# Autodesk Inventor assembly: The Final Assembly
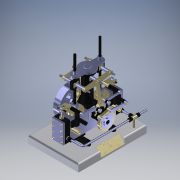
[picture p0: Inventor's stored thumbnail of the model, 180x180]
Saved by Autodesk Inventor 2016 SP1 (Build 200210100, 210)
## iProperties
Created: 2016-12-03
Part Number: The Final Assembly
Document SubType Name: Assembly
Designer: Muhammad
Author: Muhammad
## Documents named in this file (45)
- E:\Brenays Steam Engine, USB\The Final Assembly.iam
- E:\Brenays Steam Engine, USB\Base.ipt
- E:\Brenays Steam Engine, USB\Etichetta.ipt
- E:\Brenays Steam Engine, USB\Coperchio inferiore.ipt
- E:\Brenays Steam Engine, USB\Carcassa.ipt
- E:\Brenays Steam Engine, USB\Distributore.ipt
- E:\Brenays Steam Engine, USB\Coperchio.ipt
- E:\Brenays Steam Engine, USB\Premistoppa M10x1.ipt
- E:\Brenays Steam Engine, USB\Albero a gomito.ipt
- E:\Brenays Steam Engine, USB\Guida testa a croce.ipt
- E:\Brenays Steam Engine, USB\Coperchio Superiore.ipt
- E:\Brenays Steam Engine, USB\Supporto SX.ipt
- E:\Brenays Steam Engine, USB\Supporto DX.ipt
- E:\Brenays Steam Engine, USB\Asta cassetto.ipt
- E:\Brenays Steam Engine, USB\Cassetto.ipt
- E:\Brenays Steam Engine, USB\Fermo 5 mm.ipt
- E:\Brenays Steam Engine, USB\Asta cassetto_MIR.ipt
- E:\Brenays Steam Engine, USB\Cassetto_MIR.ipt
- E:\Brenays Steam Engine, USB\Fermo 5 mm_MIR.ipt
- E:\Brenays Steam Engine, USB\Biella.ipt
- E:\Brenays Steam Engine, USB\Bielletta.ipt
- E:\Brenays Steam Engine, USB\Spina cilindrica.ipt
- E:\Brenays Steam Engine, USB\Manovella.ipt
- E:\Brenays Steam Engine, USB\Assieme eccentrico.ipt
- E:\Brenays Steam Engine, USB\Testata Superiore.ipt
- E:\Brenays Steam Engine, USB\Premistoppa.ipt
- E:\Brenays Steam Engine, USB\Asta pistone.ipt
- E:\Brenays Steam Engine, USB\T di connessione1.ipt
- E:\Brenays Steam Engine, USB\Semi albero F.ipt
- E:\Brenays Steam Engine, USB\Semi alberto M.ipt
- E:\Brenays Steam Engine, USB\Traversa.ipt
- E:\Brenays Steam Engine, USB\Cursore.ipt
- E:\Brenays Steam Engine, USB\Spina cilindrica4.ipt
- E:\Brenays Steam Engine, USB\Forcella.ipt
- E:\Brenays Steam Engine, USB\Volano.ipt
- E:\Brenays Steam Engine, USB\Semi Cuscinetto.ipt
- E:\Brenays Steam Engine, USB\Varia.ipt
- E:\Brenays Steam Engine, USB\Inlet Pipe Nipple.ipt
- E:\Brenays Steam Engine, USB\Tube.ipt
- E:\Brenays Steam Engine, USB\Steam Inlet Pipe 1.ipt
- E:\Brenays Steam Engine, USB\Steam Inlet T Connector.ipt
- E:\Brenays Steam Engine, USB\M8x6 Pipe Nut.ipt
- E:\Brenays Steam Engine, USB\Exhaust Pipe Connector.ipt
- E:\Brenays Steam Engine, USB\Nut.ipt
- E:\Brenays Steam Engine, USB\Nut_MIR.ipt
## Components (93 placed, 44 different names)
1. Base:1 — Rigid:1, Rigid:2, Rigid:3, Flush:7
2. Etichetta:1 — Rigid:1
3. Coperchio inferiore:1 — Rigid:2
4. Coperchio inferiore:2 — Rigid:3, Rigid:4
5. Carcassa:1 — Rigid:4, Rigid:5, Rigid:6, Rotational:1, Rigid:11, Rigid:13, Rigid:14, Rigid:20, Rigid:21, Rigid:37, Rigid:38
6. Distributore:1 — Rigid:5, Rigid:8, Rigid:9, Rigid:26
7. Distributore:2 — Rigid:6, Rigid:7, Rigid:10, Angle:1, Mate:5, Rigid:27
8. Coperchio:1 — Rigid:7, Rigid:45, Rigid:46, Rigid:47, Rigid:48, Rigid:49, Rigid:50, Rigid:51, Rigid:52
9. Coperchio:2 — Rigid:8
10. Premistoppa M10x1:1 — Rigid:9, Mate:9
11. Premistoppa M10x1:2 — Rigid:10, Mate:1
12. Albero a gomito:1 — Rotational:1, Mate:18, Flush:4, Angle:2, Mate:28, Mate:29, Mate:30, Mate:31, Rigid:24, Mate:45, Mate:46, Mate:48, Mate:49
13. Guida testa a croce:1 — Rigid:11, Rigid:12, Mate:40
14. Coperchio Superiore:1 — Rigid:12, Mate:26, Mate:27
15. Supporto SX:1 — Rigid:14, Mate:23, Mate:55, Mate:56
16. Supporto DX:1 — Rigid:13, Rigid:19, Mate:17, Mate:24, Rotational:2
17. Asta cassetto:1 — Mate:1, Mate:4, Flush:1, Mate:44
18. Cassetto:1 — Mate:2, Rigid:15, Mate:3, Rigid:16, Angle:1, Mate:5
19. Fermo 5 mm:1 — Mate:2, Rigid:15, Mate:4
20. Fermo 5 mm:2 — Mate:3, Rigid:16, Flush:1
21. Asta cassetto_MIR:1 — Mate:6, Flush:3, Mate:9, Rigid:25
22. Cassetto_MIR:1 — Mate:7, Mate:8, Rigid:17, Rigid:18
23. Fermo 5 mm_MIR:1 — Mate:6, Mate:7, Rigid:17
24. Fermo 5 mm_MIR:2 — Flush:3, Mate:8, Rigid:18
25. Biella:1 — Mate:10, Mate:11, Mate:12, Rigid:43
26. Biella:2 — Mate:15, Mate:16, Mate:17, Mate:24, Angle:7, Rigid:44
27. Bielletta:1 — Mate:13, Mate:14, Mate:15, Mate:16, Rigid:36
28. Bielletta:2 — Mate:19, Mate:20, Mate:21, Mate:22, Rotational:4
29. Spina cilindrica:1 — Rigid:19, Mate:12
30. Assieme eccentrico:1 — Mate:18, Flush:4, Mate:25, Angle:2
31. Manovella:1 — Mate:10, Mate:11, Mate:13, Mate:14, Mate:19, Mate:20, Mate:25, Rigid:35
32. Biella:3 — Mate:21, Mate:22, Mate:23, Angle:8, Rigid:41
33. Testata Superiore:1 — Rigid:21, Rigid:23
34. Testata Superiore:2 — Rigid:20, Rigid:22
35. Premistoppa:1 — Rigid:23
36. Premistoppa:2 — Rigid:22
37. Asta pistone:1 — Mate:26, Angle:4, Angle:5, Mate:52, Flush:5
38. Asta pistone:2 — Mate:27, Angle:4, Mate:54, Flush:6
39. T di connessione1:1 — Mate:28, Mate:29, Mate:32, Angle:3, Mate:35, Mate:36, Mate:37, Angle:5, Mate:41, Mate:42, Mate:47
40. T di connessione1:2 — Mate:30, Mate:31, Mate:33, Angle:3, Mate:34, Mate:38, Mate:39, Mate:50
41. Semi albero F:1 — Mate:33, Mate:34
42. Semi alberto M:1 — Mate:32, Mate:35, Mate:51
43. Semi alberto M:2 — Mate:36, Mate:37, Mate:53
44. Semi albero F:2 — Mate:38, Mate:39
45. Traversa:1 — Mate:41, Mate:42, Mate:43
46. Cursore:1 — Mate:40, Mate:43
47. Spina cilindrica4:1 — Mate:44, Angle:6
48. Forcella:1 — Rotational:2, Angle:6, Angle:7
49. Volano:1 — Rigid:24
50. Semi Cuscinetto:1 — Mate:45, Mate:46, Mate:47
51. Semi Cuscinetto:2 — Mate:48, Mate:49, Mate:50
52. Varia:1 — Mate:51, Mate:52, Flush:5
53. Varia:2 — Mate:53, Mate:54, Flush:6
54. Forcella:2 — Mate:55, Mate:56, Angle:8
55. Spina cilindrica4:2 — Rigid:25
56. Inlet Pipe Nipple:1 — Rigid:26, Rotational:3, Rigid:30
57. Inlet Pipe Nipple:2 — Rigid:27, Rigid:28, Rigid:33
58. Tube:1 — Rotational:3, Mate:57
59. Steam Inlet Pipe 1:1 — Rigid:28, Mate:58
60. Steam Inlet T Connector:1 — Mate:57, Mate:58, Rigid:29, Rigid:31, Rigid:32, Rigid:34
61. Steam Inlet Pipe 1:2 — Rigid:29
62. M8x6 Pipe Nut:1 — Rigid:34
63. M8x6 Pipe Nut:2 — Rigid:32
64. M8x6 Pipe Nut:3 — Rigid:31
65. M8x6 Pipe Nut:4 — Rigid:30
66. M8x6 Pipe Nut:5 — Rigid:33
67. Fermo 5 mm:3 — Rigid:35, Rigid:42
68. Fermo 5 mm:4 — Rotational:4, Rigid:40
69. Fermo 5 mm:5 — Rigid:36, Rigid:39
70. Exhaust Pipe Connector:1 — Rigid:37
71. Exhaust Pipe Connector:2 — Rigid:38
72. Spina cilindrica:2 — Rigid:39
73. Spina cilindrica:3 — Rigid:41
74. Spina cilindrica:4 — Rigid:40
75. Spina cilindrica:5 — Rigid:43
76. Spina cilindrica:6 — Rigid:42
77. Spina cilindrica:7 — Rigid:44
78. Nut:6 — Rigid:45
79. Nut:7 — Rigid:46
80. Nut:8 — Rigid:47
81. Nut:9 — Rigid:48
82. Nut:10 — Rigid:49
83. Nut:11 — Rigid:50
84. Nut:12 — Rigid:51
85. Nut:13 — Rigid:52
86. Nut_MIR:1
87. Nut_MIR:2
88. Nut_MIR:3
89. Nut_MIR:4
90. Nut_MIR:5
91. Nut_MIR:6
92. Nut_MIR:7
93. Nut_MIR:8
## Relationships (129: Mate 58, WeldJoint 52, Angle 8, Flush 7, RevoluteJoint 4)
- Rigid:1 [WeldJoint]: Base:1 ↔ Etichetta:1
- Rigid:2 [WeldJoint]: Base:1 ↔ Coperchio inferiore:1
- Rigid:3 [WeldJoint]: Base:1 ↔ Coperchio inferiore:2
- Rigid:4 [WeldJoint]: Coperchio inferiore:2 ↔ Carcassa:1
- Rigid:5 [WeldJoint]: Carcassa:1 ↔ Distributore:1
- Rigid:6 [WeldJoint]: Carcassa:1 ↔ Distributore:2
- Rigid:7 [WeldJoint]: Distributore:2 ↔ Coperchio:1
- Rigid:8 [WeldJoint]: Distributore:1 ↔ Coperchio:2
- Rigid:9 [WeldJoint]: Distributore:1 ↔ Premistoppa M10x1:1
- Rigid:10 [WeldJoint]: Distributore:2 ↔ Premistoppa M10x1:2
- Rotational:1 [RevoluteJoint]: Carcassa:1 ↔ Albero a gomito:1
- Rigid:11 [WeldJoint]: Carcassa:1 ↔ Guida testa a croce:1
- Rigid:12 [WeldJoint]: Guida testa a croce:1 ↔ Coperchio Superiore:1
- Rigid:13 [WeldJoint]: Carcassa:1 ↔ Supporto DX:1
- Rigid:14 [WeldJoint]: Carcassa:1 ↔ Supporto SX:1
- Mate:1: Premistoppa M10x1:2 ↔ Asta cassetto:1
- Mate:2: Cassetto:1 ↔ Fermo 5 mm:1
- Rigid:15 [WeldJoint]: Cassetto:1 ↔ Fermo 5 mm:1
- Mate:3: Cassetto:1 ↔ Fermo 5 mm:2
- Rigid:16 [WeldJoint]: Cassetto:1 ↔ Fermo 5 mm:2
- Mate:4: Asta cassetto:1 ↔ Fermo 5 mm:1
- Angle:1 (0 deg): Distributore:2 ↔ Cassetto:1
- Mate:5: Distributore:2 ↔ Cassetto:1
- Flush:1 (1.7 mm): Asta cassetto:1 ↔ Fermo 5 mm:2
- Flush:2
- Mate:6: Asta cassetto_MIR:1 ↔ Fermo 5 mm_MIR:1
- Mate:7: Cassetto_MIR:1 ↔ Fermo 5 mm_MIR:1
- Flush:3 (1.7 mm): Asta cassetto_MIR:1 ↔ Fermo 5 mm_MIR:2
- Mate:8: Cassetto_MIR:1 ↔ Fermo 5 mm_MIR:2
- Rigid:17 [WeldJoint]: Cassetto_MIR:1 ↔ Fermo 5 mm_MIR:1
- Rigid:18 [WeldJoint]: Cassetto_MIR:1 ↔ Fermo 5 mm_MIR:2
- Mate:9: Premistoppa M10x1:1 ↔ Asta cassetto_MIR:1
- Rigid:19 [WeldJoint]: Supporto DX:1 ↔ Spina cilindrica:1
- Mate:10: Biella:1 ↔ Manovella:1
- Mate:11: Biella:1 ↔ Manovella:1
- Mate:12: Biella:1 ↔ Spina cilindrica:1
- Mate:13: Bielletta:1 ↔ Manovella:1
- Mate:14: Bielletta:1 ↔ Manovella:1
- Mate:15: Biella:2 ↔ Bielletta:1
- Mate:16: Biella:2 ↔ Bielletta:1
- Mate:17: Supporto DX:1 ↔ Biella:2
- Mate:18: Albero a gomito:1 ↔ Assieme eccentrico:1
- Mate:19: Bielletta:2 ↔ Manovella:1
- Mate:20: Bielletta:2 ↔ Manovella:1
- Mate:21: Bielletta:2 ↔ Biella:3
- Mate:22: Bielletta:2 ↔ Biella:3
- Mate:23: Supporto SX:1 ↔ Biella:3
- Mate:24: Supporto DX:1 ↔ Biella:2
- Flush:4: Albero a gomito:1 ↔ Assieme eccentrico:1
- Mate:25: Assieme eccentrico:1 ↔ Manovella:1
- Angle:2 (0 deg): Albero a gomito:1 ↔ Assieme eccentrico:1
- Rigid:20 [WeldJoint]: Carcassa:1 ↔ Testata Superiore:2
- Rigid:21 [WeldJoint]: Carcassa:1 ↔ Testata Superiore:1
- Rigid:22 [WeldJoint]: Testata Superiore:2 ↔ Premistoppa:2
- Rigid:23 [WeldJoint]: Testata Superiore:1 ↔ Premistoppa:1
- Mate:26: Coperchio Superiore:1 ↔ Asta pistone:1
- Mate:27: Coperchio Superiore:1 ↔ Asta pistone:2
- Mate:28: Albero a gomito:1 ↔ T di connessione1:1
- Mate:29: Albero a gomito:1 ↔ T di connessione1:1
- Mate:30: Albero a gomito:1 ↔ T di connessione1:2
- Mate:31: Albero a gomito:1 ↔ T di connessione1:2
- Mate:32: T di connessione1:1 ↔ Semi alberto M:1
- Mate:33: T di connessione1:2 ↔ Semi albero F:1
- Angle:3 (0 deg): T di connessione1:1 ↔ T di connessione1:2
- Mate:34: T di connessione1:2 ↔ Semi albero F:1
- Mate:35: T di connessione1:1 ↔ Semi alberto M:1
- Mate:36: T di connessione1:1 ↔ Semi alberto M:2
- Mate:37: T di connessione1:1 ↔ Semi alberto M:2
- Mate:38: T di connessione1:2 ↔ Semi albero F:2
- Mate:39: T di connessione1:2 ↔ Semi albero F:2
- Angle:4 (0 deg): Asta pistone:1 ↔ Asta pistone:2
- Angle:5 (0 deg): Asta pistone:1 ↔ T di connessione1:1
- Mate:40: Guida testa a croce:1 ↔ Cursore:1
- Mate:41: T di connessione1:1 ↔ Traversa:1
- Mate:42: T di connessione1:1 ↔ Traversa:1
- Mate:43: Traversa:1 ↔ Cursore:1
- Mate:44: Asta cassetto:1 ↔ Spina cilindrica4:1
- Rotational:2 [RevoluteJoint]: Supporto DX:1 ↔ Forcella:1
- Angle:6 (0 deg): Spina cilindrica4:1 ↔ Forcella:1
- Rigid:24 [WeldJoint]: Albero a gomito:1 ↔ Volano:1
- Mate:45: Albero a gomito:1 ↔ Semi Cuscinetto:1
- Mate:46: Albero a gomito:1 ↔ Semi Cuscinetto:1
- Mate:47: T di connessione1:1 ↔ Semi Cuscinetto:1
- Mate:48: Albero a gomito:1 ↔ Semi Cuscinetto:2
- Mate:49: Albero a gomito:1 ↔ Semi Cuscinetto:2
- Mate:50: T di connessione1:2 ↔ Semi Cuscinetto:2
- Angle:7 (0 deg): Biella:2 ↔ Forcella:1
- Mate:51: Semi alberto M:1 ↔ Varia:1
- Mate:52: Asta pistone:1 ↔ Varia:1
- Mate:53: Semi alberto M:2 ↔ Varia:2
- Mate:54: Asta pistone:2 ↔ Varia:2
- Flush:5 (-0.25 mm): Asta pistone:1 ↔ Varia:1
- Flush:6 (-0.25 mm): Asta pistone:2 ↔ Varia:2
- Rigid:25 [WeldJoint]: Asta cassetto_MIR:1 ↔ Spina cilindrica4:2
- Mate:55: Supporto SX:1 ↔ Forcella:2
- Mate:56: Supporto SX:1 ↔ Forcella:2
- Angle:8 (0 deg): Biella:3 ↔ Forcella:2
- Rigid:26 [WeldJoint]: Distributore:1 ↔ Inlet Pipe Nipple:1
- Rigid:27 [WeldJoint]: Distributore:2 ↔ Inlet Pipe Nipple:2
- Rotational:3 [RevoluteJoint]: Inlet Pipe Nipple:1 ↔ Tube:1
- Rigid:28 [WeldJoint]: Inlet Pipe Nipple:2 ↔ Steam Inlet Pipe 1:1
- Mate:57: Tube:1 ↔ Steam Inlet T Connector:1
- Mate:58: Steam Inlet Pipe 1:1 ↔ Steam Inlet T Connector:1
- Rigid:29 [WeldJoint]: Steam Inlet T Connector:1 ↔ Steam Inlet Pipe 1:2
- Rigid:30 [WeldJoint]: Inlet Pipe Nipple:1 ↔ M8x6 Pipe Nut:4
- Rigid:31 [WeldJoint]: Steam Inlet T Connector:1 ↔ M8x6 Pipe Nut:3
- Rigid:32 [WeldJoint]: Steam Inlet T Connector:1 ↔ M8x6 Pipe Nut:2
- Rigid:33 [WeldJoint]: Inlet Pipe Nipple:2 ↔ M8x6 Pipe Nut:5
- Rigid:34 [WeldJoint]: Steam Inlet T Connector:1 ↔ M8x6 Pipe Nut:1
- Flush:7 (300 mm): Base:1
- Rigid:35 [WeldJoint]: Manovella:1 ↔ Fermo 5 mm:3
- Rigid:36 [WeldJoint]: Bielletta:1 ↔ Fermo 5 mm:5
- Rotational:4 [RevoluteJoint]: Bielletta:2 ↔ Fermo 5 mm:4
- Rigid:37 [WeldJoint]: Carcassa:1 ↔ Exhaust Pipe Connector:1
- Rigid:38 [WeldJoint]: Carcassa:1 ↔ Exhaust Pipe Connector:2
- Rigid:39 [WeldJoint]: Fermo 5 mm:5 ↔ Spina cilindrica:2
- Rigid:40 [WeldJoint]: Fermo 5 mm:4 ↔ Spina cilindrica:4
- Rigid:41 [WeldJoint]: Biella:3 ↔ Spina cilindrica:3
- Rigid:42 [WeldJoint]: Fermo 5 mm:3 ↔ Spina cilindrica:6
- Rigid:43 [WeldJoint]: Biella:1 ↔ Spina cilindrica:5
- Rigid:44 [WeldJoint]: Biella:2 ↔ Spina cilindrica:7
- Rigid:45 [WeldJoint]: Coperchio:1 ↔ Nut:6
- Rigid:46 [WeldJoint]: Coperchio:1 ↔ Nut:7
- Rigid:47 [WeldJoint]: Coperchio:1 ↔ Nut:8
- Rigid:48 [WeldJoint]: Coperchio:1 ↔ Nut:9
- Rigid:49 [WeldJoint]: Coperchio:1 ↔ Nut:10
- Rigid:50 [WeldJoint]: Coperchio:1 ↔ Nut:11
- Rigid:51 [WeldJoint]: Coperchio:1 ↔ Nut:12
- Rigid:52 [WeldJoint]: Coperchio:1 ↔ Nut:13
